# Autodesk Inventor assembly: ensamblado
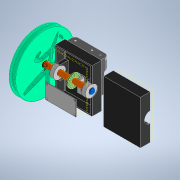
[picture p0: Inventor's stored thumbnail of the model, 180x180]
Saved by Autodesk Inventor 2021 (Build 250183000, 183)
## iProperties
Created: 2021-12-11
Part Number: ensamblado
Document SubType Name: Assembly
Designer: Juan M. Casillas
Author: Juan M. Casillas
## Documents named in this file (13)
- K:\3DPrinting\3DModels\3party\ElectricEel_rueca\medidor\ensamblado.iam
- K:\3DPrinting\3DModels\3party\ElectricEel_rueca\medidor\carrete.ipt
- K:\3DPrinting\3DModels\3party\ElectricEel_rueca\medidor\eje_solo.ipt
- K:\3DPrinting\3DModels\3party\ElectricEel_rueca\medidor\separador_20.ipt
- K:\3DPrinting\3DModels\3party\ElectricEel_rueca\medidor\rodamiento.ipt
- K:\3DPrinting\3DModels\3party\ElectricEel_rueca\medidor\encoder.ipt
- K:\3DPrinting\3DModels\3party\ElectricEel_rueca\medidor\separador_15.ipt
- K:\3DPrinting\3DModels\3party\ElectricEel_rueca\medidor\rosca.ipt
- K:\3DPrinting\3DModels\3party\ElectricEel_rueca\medidor\cierre.ipt
- K:\3DPrinting\3DModels\3party\ElectricEel_rueca\medidor\caja_base.ipt
- K:\3DPrinting\3DModels\CatFeeder\Case\version6\esp32_footprint.ipt
- K:\3DPrinting\3DModels\3party\ElectricEel_rueca\medidor\irencoder_footprint.ipt
- K:\3DPrinting\3DModels\3party\battery holder\User Library-R6_AA_UM3-1_5V_holder4AA.ipt
## Components (17 placed, 12 different names)
1. carrete:1 — Mate:4, Mate:7
2. eje_solo:1 — Mate:3, Mate:4, Mate:5, Mate:9
3. separador_20:1 — Mate:7
4. rodamiento:1 — Mate:1, Mate:8
5. rodamiento:2 — Mate:2, Mate:3, Mate:10, Mate:11
6. encoder:1 — Mate:12
7. separador_15:1 — Mate:8
8. separador_15:2 — Mate:11, Mate:12
9. rosca:1 — Mate:5, Mate:6
10. rosca:2 — Mate:9
11. cierre:1 — Mate:10
12. cierre:2 — Mate:6
13. caja_base:1 — Mate:1, Mate:2
14. irencoder_footprint:1
15. esp32_footprint:1
16. User Library-R6_AA_UM3-1_5V_holder4AA:1
17. caja_base:2
## Relationships (12: Mate 12)
- Mate:1: rodamiento:1 ↔ caja_base:1
- Mate:2: rodamiento:2 ↔ caja_base:1
- Mate:3: eje_solo:1 ↔ rodamiento:2
- Mate:4: carrete:1 ↔ eje_solo:1
- Mate:5: eje_solo:1 ↔ rosca:1
- Mate:6: rosca:1 ↔ cierre:2
- Mate:7: carrete:1 ↔ separador_20:1
- Mate:8: rodamiento:1 ↔ separador_15:1
- Mate:9: eje_solo:1 ↔ rosca:2
- Mate:10: rodamiento:2 ↔ cierre:1
- Mate:11: rodamiento:2 ↔ separador_15:2
- Mate:12: encoder:1 ↔ separador_15:2
